# Autodesk Inventor assembly: Сборка
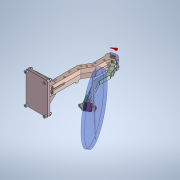
[picture p0: Inventor's stored thumbnail of the model, 180x180]
Saved by Autodesk Inventor 2021.2 (Build 252289000, 289)
## iProperties
Created: 2024-10-29
Part Number: Сборка
Document SubType Name: Assembly
Designer: barko
Mass: 1383.59 g
Surface Area: 2828.64 cm^2
Volume: 1218.78 cm^3
Density: 1.13522 g/cm^3
Author: barko
## Documents named in this file (30)
- C:\Users\barko\Desktop\Daniil\MIET\PID_controller\Mechanics\3D_model\Сборка.iam
- C:\Users\barko\Desktop\Daniil\MIET\PID_controller\Mechanics\3D_model\Детали твёрдого тела\Ножка 1.ipt
- C:\Users\barko\Desktop\Daniil\MIET\PID_controller\Mechanics\3D_model\Детали твёрдого тела\Ножка 2.ipt
- C:\Users\barko\Desktop\Daniil\MIET\PID_controller\Mechanics\3D_model\Детали твёрдого тела\Скобка 1.ipt
- C:\Users\barko\Desktop\Daniil\MIET\PID_controller\Mechanics\3D_model\Детали твёрдого тела\Скобка 2.ipt
- C:\Users\barko\Desktop\Daniil\MIET\PID_controller\Mechanics\3D_model\Детали твёрдого тела\Фланец.ipt
- C:\Users\barko\Desktop\Daniil\MIET\PID_controller\Mechanics\3D_model\Детали твёрдого тела\Луч.ipt
- C:\Users\barko\Desktop\Daniil\MIET\PID_controller\Mechanics\3D_model\Детали твёрдого тела\Ложечка.ipt
- C:\Users\barko\Desktop\Daniil\MIET\PID_controller\Mechanics\3D_model\Моторчик.ipt
- C:\Users\barko\Desktop\Daniil\MIET\PID_controller\Mechanics\3D_model\Пропеллер.ipt
- C:\Users\barko\Documents\Inventor\Content Center Files\R2021\ru-RU\Nut GOST 15524-70\Гайка M4-6H ГОСТ 15524-70.ipt
- C:\Users\barko\Documents\Inventor\Content Center Files\R2021\ru-RU\GOST 11738-84\Винт M4-6gx20 ГОСТ 11738-84.ipt
- C:\Users\barko\Desktop\Daniil\MIET\PID_controller\Mechanics\3D_model\Подшипник.ipt
- C:\Users\barko\Documents\Inventor\Content Center Files\R2021\ru-RU\GOST 5915-70\Гайка M6-6H ГОСТ 5915-70(1).ipt
- C:\Users\barko\Documents\Inventor\Content Center Files\R2021\ru-RU\GOST 11738-84\Винт M6-6gx50 ГОСТ 11738-84.ipt
- C:\Users\barko\Documents\Inventor\Content Center Files\R2021\ru-RU\GOST 11371-78  A\Шайба 6 ГОСТ 11371-78.ipt
- C:\Users\barko\Documents\Inventor\Content Center Files\R2021\ru-RU\Washer 1 GOST 6402-78\Шайба 6Л ГОСТ 6402-78.ipt
- C:\Users\barko\Documents\Inventor\Content Center Files\R2021\ru-RU\GOST 17475-80 (2)\Винт 2.M6-6gx30 ГОСТ 17475-80.ipt
- C:\Users\barko\Documents\Inventor\Content Center Files\R2021\ru-RU\ISO 10642(1)\ISO 10642 - M3x8.ipt
- C:\Users\barko\Documents\Inventor\Content Center Files\R2021\ru-RU\ISO 10642(1)\ISO 10642 - M3x12.ipt
- C:\Users\barko\Desktop\Daniil\MIET\PID_controller\Mechanics\3D_model\Детали твёрдого тела\Вал насадка 1.ipt
- C:\Users\barko\Desktop\Daniil\MIET\PID_controller\Mechanics\3D_model\Метизы\Гайка M4-6H ГОСТ 11860-85.ipt
- C:\Users\barko\Desktop\Daniil\MIET\PID_controller\Mechanics\3D_model\Метизы\Шайба A 4 ГОСТ 6958-78.ipt
- C:\Users\barko\Desktop\Daniil\MIET\PID_controller\Mechanics\3D_model\Стрелочка.ipt
- C:\Users\barko\Documents\Inventor\Content Center Files\R2021\ru-RU\GOST 11738-84\Винт M4-6gx25 ГОСТ 11738-84.ipt
- C:\Users\barko\Documents\Inventor\Content Center Files\R2021\ru-RU\GOST 11738-84\Винт M6-6gx30 ГОСТ 11738-84.ipt
- C:\Users\barko\Desktop\Daniil\MIET\PID_controller\Mechanics\3D_model\Детали твёрдого тела\Вал стержень.ipt
- C:\Users\barko\Desktop\Daniil\MIET\PID_controller\Mechanics\3D_model\Детали твёрдого тела\Блок.ipt
- C:\Users\barko\Documents\Inventor\Content Center Files\R2021\ru-RU\GOST 11738-84\Винт M3-6gx30 ГОСТ 11738-84.ipt
- C:\Users\barko\Documents\Inventor\Content Center Files\R2021\ru-RU\GOST 5916-70\Гайка M3-6H ГОСТ 5916-70.ipt
## Components (78 placed, 29 different names)
1. Ножка 1:1 — Совмещение:1, Угол:1, Совмещение:62, Совмещение:64, Вставка:26, Совмещение:100, Совмещение:101, Совмещение:102, Совмещение:105, Совмещение:106, Совмещение:107, Совмещение:127, Совмещение:128, Совмещение:129, Совмещение:130, Совмещение:131, Совмещение:132, Совмещение:133, Совмещение:134, Совмещение:135, Совмещение:136, Совмещение:137, Совмещение:138, Совмещение:139, Совмещение:140, Совмещение:141, Совмещение:142, Совмещение:143, Совмещение:144, Совмещение:145, Совмещение:147, Совмещение:149, Совмещение:151, Совмещение:153, Совмещение:155, Совмещение:157, Совмещение:159, Совмещение:161
2. Ножка 2:1 — Совмещение:63, Совмещение:65, Совмещение:115, Совмещение:116, Совмещение:117, Совмещение:121, Совмещение:122, Совмещение:123, Совмещение:146, Совмещение:148, Совмещение:150, Совмещение:152, Совмещение:154, Совмещение:156, Совмещение:158, Совмещение:160, Совмещение:162
3. Скобка 1:1 — Совмещение:104, Совмещение:109
4. Скобка 2:1 — Совмещение:119, Совмещение:120
5. Фланец:1 — Совмещение:66, Совмещение:67, Совмещение:68, Совмещение:69, Совмещение:70, Совмещение:71, Совмещение:72, Совмещение:73, Совмещение:74, Совмещение:75, Совмещение:76, Совмещение:77, Вставка:6, Вставка:7, Вставка:8, Вставка:9, Заподлицо:2, Заподлицо:3, Заподлицо:4, Заподлицо:5
6. Луч:1 — Заподлицо:1, Совмещение:1, Угол:1, Совмещение:96, Угол:2, Совмещение:97, Заподлицо:6, Угол:3, Совмещение:110, Совмещение:111, Совмещение:112, Совмещение:114
7. Ложечка:1 — Совмещение:87, Совмещение:88, Совмещение:91, Совмещение:92, Совмещение:93, Совмещение:94, Совмещение:96, Угол:2, Совмещение:97, Заподлицо:6, Совмещение:98, Совмещение:99
8. Моторчик:1 — Вставка:2, Совмещение:98, Совмещение:99
9. Пропеллер:1 — Вставка:2
10. Подшипник:1 — Вставка:25, Вставка:26, Вставка:29
11. Подшипник:2 — Вставка:32, Вставка:34
12. Вал насадка 1:1 — Вставка:25, Вставка:32, Совмещение:125
13. Гайка M4-6H ГОСТ 11860-85:2
14. Стрелочка:1 — Угол:3
15. Шайба A 4 ГОСТ 6958-78:3 — Вставка:29, Вставка:33
16. Вал стержень:1 — Совмещение:125, Заподлицо:7
17. Гайка ГОСТ 15524-70 M4:6 — Вставка:33, Заподлицо:7
18. Блок:1 — Вставка:35, Вставка:36, Совмещение:126
19. Шайба A 4 ГОСТ 6958-78:4 — Вставка:34, Вставка:35
20. Гайка ГОСТ 15524-70 M4:7 — Вставка:36, Совмещение:126
21. Гайка ГОСТ 5916-70 M3:9 — Совмещение:161, Совмещение:162
22. Гайка ГОСТ 5916-70 M3:8 — Совмещение:159, Совмещение:160
23. Гайка ГОСТ 5916-70 M3:7 — Совмещение:157, Совмещение:158
24. Гайка ГОСТ 5916-70 M3:6 — Совмещение:155, Совмещение:156
25. Гайка ГОСТ 5916-70 M3:5 — Совмещение:153, Совмещение:154
26. Гайка ГОСТ 5916-70 M3:4 — Совмещение:151, Совмещение:152
27. Гайка ГОСТ 5916-70 M3:3 — Совмещение:149, Совмещение:150
28. Гайка ГОСТ 5916-70 M3:2 — Совмещение:147, Совмещение:148
29. Винт ГОСТ 11738-84 M 3x30:9 — Совмещение:143, Совмещение:144
30. Винт ГОСТ 11738-84 M 3x30:8 — Совмещение:141, Совмещение:142
31. Винт ГОСТ 11738-84 M 3x30:7 — Совмещение:139, Совмещение:140
32. Винт ГОСТ 11738-84 M 3x30:6 — Совмещение:137, Совмещение:138
33. Винт ГОСТ 11738-84 M 3x30:5 — Совмещение:135, Совмещение:136
34. Винт ГОСТ 11738-84 M 3x30:4 — Совмещение:133, Совмещение:134
35. Винт ГОСТ 11738-84 M 3x30:3 — Совмещение:131, Совмещение:132
36. Винт ГОСТ 11738-84 M 3x30:2 — Совмещение:129, Совмещение:130
37. Гайка ГОСТ 5916-70 M3:1 — Совмещение:145, Совмещение:146
38. Винт ГОСТ 11738-84 M 3x30:1 — Совмещение:127, Совмещение:128
39. Винт ГОСТ 11738-84 M 4x25:1 — Совмещение:103, Совмещение:104
40. Гайка ГОСТ 15524-70 M4:1 — Совмещение:100, Совмещение:101, Совмещение:102, Совмещение:103
41. Винт ГОСТ 11738-84 M 4x25:2 — Совмещение:113, Совмещение:114
42. Гайка ГОСТ 15524-70 M4:2 — Совмещение:110, Совмещение:111, Совмещение:112, Совмещение:113
43. Винт ГОСТ 11738-84 M 4x20:2 — Совмещение:108, Совмещение:109
44. Винт ГОСТ 11738-84 M 4x25:3 — Совмещение:118, Совмещение:119
45. Винт ГОСТ 11738-84 M 4x20:4 — Совмещение:120, Совмещение:124
46. Гайка ГОСТ 15524-70 M4:3 — Совмещение:115, Совмещение:116, Совмещение:117, Совмещение:118
47. Гайка ГОСТ 15524-70 M4:4 — Совмещение:105, Совмещение:106, Совмещение:107, Совмещение:108
48. Гайка ГОСТ 15524-70 M4:5 — Совмещение:121, Совмещение:122, Совмещение:123, Совмещение:124
49. Гайка ГОСТ 5915-70 M6:1 — Совмещение:69, Совмещение:72, Совмещение:73, Совмещение:80
50. Гайка ГОСТ 5915-70 M6:2 — Совмещение:71, Совмещение:74, Совмещение:75, Совмещение:81
51. Гайка ГОСТ 5915-70 M6:3 — Совмещение:70, Совмещение:76, Совмещение:77, Совмещение:79
52. Гайка ГОСТ 5915-70 M6:4 — Совмещение:66, Совмещение:67, Совмещение:68, Совмещение:78
53. Винт ГОСТ 11738-84 M 6x50:1 — Совмещение:64, Совмещение:79
54. Винт ГОСТ 11738-84 M 6x30:1 — Совмещение:63, Совмещение:80
55. Винт ГОСТ 11738-84 M 6x30:2 — Совмещение:62, Совмещение:78
56. Винт ГОСТ 11738-84 M 6x50:2 — Совмещение:65, Совмещение:81
57. Шайба  ГОСТ 11371-78 6,4:1 — Вставка:6, Вставка:10
58. Шайба  ГОСТ 11371-78 6,4:2 — Вставка:7, Вставка:11
59. Шайба  ГОСТ 11371-78 6,4:3 — Вставка:8, Вставка:13
60. Шайба  ГОСТ 11371-78 6,4:4 — Вставка:9, Вставка:12
61. Шайба 1 ГОСТ 6402-78 6Л:1 — Вставка:10, Вставка:16
62. Шайба 1 ГОСТ 6402-78 6Л:2 — Вставка:11, Вставка:15
63. Шайба 1 ГОСТ 6402-78 6Л:3 — Вставка:12, Вставка:17
64. Шайба 1 ГОСТ 6402-78 6Л:4 — Вставка:13, Вставка:14
65. Гайка ГОСТ 5915-70 M6:5 — Вставка:14, Совмещение:85
66. Гайка ГОСТ 5915-70 M6:6 — Вставка:15, Совмещение:84
67. Гайка ГОСТ 5915-70 M6:7 — Вставка:16, Совмещение:82
68. Гайка ГОСТ 5915-70 M6:8 — Вставка:17, Совмещение:83
69. Винт 2 ГОСТ 17475-80 M6 x 30:1 — Совмещение:82, Заподлицо:3
70. Винт 2 ГОСТ 17475-80 M6 x 30:2 — Совмещение:83, Заподлицо:2
71. Винт 2 ГОСТ 17475-80 M6 x 30:3 — Совмещение:85, Заподлицо:5
72. Винт 2 ГОСТ 17475-80 M6 x 30:4 — Совмещение:84, Заподлицо:4
73. ISO 10642 M3x12:2 — Совмещение:87
74. ISO 10642 M3x12:3 — Совмещение:88
75. ISO 10642 M3x8:1 — Совмещение:91
76. ISO 10642 M3x8:2 — Совмещение:92
77. ISO 10642 M3x8:3 — Совмещение:93
78. ISO 10642 M3x8:4 — Совмещение:94
## Relationships (129: Mate 98, Insert 21, Flush 7, Angle 3)
- Вставка:2 [Insert] (2 mm): Моторчик:1 ↔ Пропеллер:1
- Заподлицо:1 [Flush]: Луч:1
- Совмещение:1 [Mate]: Ножка 1:1 ↔ Луч:1
- Угол:1 [Angle] (0 deg): Ножка 1:1 ↔ Луч:1
- Совмещение:62 [Mate]: Ножка 1:1 ↔ Винт ГОСТ 11738-84 M 6x30:2
- Совмещение:63 [Mate]: Ножка 2:1 ↔ Винт ГОСТ 11738-84 M 6x30:1
- Совмещение:64 [Mate]: Ножка 1:1 ↔ Винт ГОСТ 11738-84 M 6x50:1
- Совмещение:65 [Mate]: Ножка 2:1 ↔ Винт ГОСТ 11738-84 M 6x50:2
- Совмещение:66 [Mate]: Фланец:1 ↔ Гайка ГОСТ 5915-70 M6:4
- Совмещение:67 [Mate]: Фланец:1 ↔ Гайка ГОСТ 5915-70 M6:4
- Совмещение:68 [Mate]: Фланец:1 ↔ Гайка ГОСТ 5915-70 M6:4
- Совмещение:69 [Mate]: Фланец:1 ↔ Гайка ГОСТ 5915-70 M6:1
- Совмещение:70 [Mate]: Фланец:1 ↔ Гайка ГОСТ 5915-70 M6:3
- Совмещение:71 [Mate]: Фланец:1 ↔ Гайка ГОСТ 5915-70 M6:2
- Совмещение:72 [Mate]: Фланец:1 ↔ Гайка ГОСТ 5915-70 M6:1
- Совмещение:73 [Mate]: Фланец:1 ↔ Гайка ГОСТ 5915-70 M6:1
- Совмещение:74 [Mate]: Фланец:1 ↔ Гайка ГОСТ 5915-70 M6:2
- Совмещение:75 [Mate]: Фланец:1 ↔ Гайка ГОСТ 5915-70 M6:2
- Совмещение:76 [Mate]: Фланец:1 ↔ Гайка ГОСТ 5915-70 M6:3
- Совмещение:77 [Mate]: Фланец:1 ↔ Гайка ГОСТ 5915-70 M6:3
- Совмещение:78 [Mate]: Гайка ГОСТ 5915-70 M6:4 ↔ Винт ГОСТ 11738-84 M 6x30:2
- Совмещение:79 [Mate]: Гайка ГОСТ 5915-70 M6:3 ↔ Винт ГОСТ 11738-84 M 6x50:1
- Совмещение:80 [Mate]: Гайка ГОСТ 5915-70 M6:1 ↔ Винт ГОСТ 11738-84 M 6x30:1
- Совмещение:81 [Mate]: Гайка ГОСТ 5915-70 M6:2 ↔ Винт ГОСТ 11738-84 M 6x50:2
- Вставка:6 [Insert]: Фланец:1 ↔ Шайба  ГОСТ 11371-78 6,4:1
- Вставка:7 [Insert]: Фланец:1 ↔ Шайба  ГОСТ 11371-78 6,4:2
- Вставка:8 [Insert]: Фланец:1 ↔ Шайба  ГОСТ 11371-78 6,4:3
- Вставка:9 [Insert]: Фланец:1 ↔ Шайба  ГОСТ 11371-78 6,4:4
- Вставка:10 [Insert]: Шайба  ГОСТ 11371-78 6,4:1 ↔ Шайба 1 ГОСТ 6402-78 6Л:1
- Вставка:11 [Insert]: Шайба  ГОСТ 11371-78 6,4:2 ↔ Шайба 1 ГОСТ 6402-78 6Л:2
- Вставка:12 [Insert]: Шайба  ГОСТ 11371-78 6,4:4 ↔ Шайба 1 ГОСТ 6402-78 6Л:3
- Вставка:13 [Insert]: Шайба  ГОСТ 11371-78 6,4:3 ↔ Шайба 1 ГОСТ 6402-78 6Л:4
- Вставка:14 [Insert]: Шайба 1 ГОСТ 6402-78 6Л:4 ↔ Гайка ГОСТ 5915-70 M6:5
- Вставка:15 [Insert]: Шайба 1 ГОСТ 6402-78 6Л:2 ↔ Гайка ГОСТ 5915-70 M6:6
- Вставка:16 [Insert]: Шайба 1 ГОСТ 6402-78 6Л:1 ↔ Гайка ГОСТ 5915-70 M6:7
- Вставка:17 [Insert]: Шайба 1 ГОСТ 6402-78 6Л:3 ↔ Гайка ГОСТ 5915-70 M6:8
- Совмещение:82 [Mate]: Гайка ГОСТ 5915-70 M6:7 ↔ Винт 2 ГОСТ 17475-80 M6 x 30:1
- Совмещение:83 [Mate]: Гайка ГОСТ 5915-70 M6:8 ↔ Винт 2 ГОСТ 17475-80 M6 x 30:2
- Совмещение:84 [Mate]: Гайка ГОСТ 5915-70 M6:6 ↔ Винт 2 ГОСТ 17475-80 M6 x 30:4
- Совмещение:85 [Mate]: Гайка ГОСТ 5915-70 M6:5 ↔ Винт 2 ГОСТ 17475-80 M6 x 30:3
- Заподлицо:2 [Flush] (9 mm): Фланец:1 ↔ Винт 2 ГОСТ 17475-80 M6 x 30:2
- Заподлицо:3 [Flush] (9 mm): Фланец:1 ↔ Винт 2 ГОСТ 17475-80 M6 x 30:1
- Заподлицо:4 [Flush] (9 mm): Фланец:1 ↔ Винт 2 ГОСТ 17475-80 M6 x 30:4
- Заподлицо:5 [Flush] (9 mm): Фланец:1 ↔ Винт 2 ГОСТ 17475-80 M6 x 30:3
- Совмещение:87 [Mate]: Ложечка:1 ↔ ISO 10642 M3x12:2
- Совмещение:88 [Mate]: Ложечка:1 ↔ ISO 10642 M3x12:3
- Совмещение:91 [Mate]: Ложечка:1 ↔ ISO 10642 M3x8:1
- Совмещение:92 [Mate]: Ложечка:1 ↔ ISO 10642 M3x8:2
- Совмещение:93 [Mate]: Ложечка:1 ↔ ISO 10642 M3x8:3
- Совмещение:94 [Mate]: Ложечка:1 ↔ ISO 10642 M3x8:4
- Совмещение:96 [Mate]: Луч:1 ↔ Ложечка:1
- Угол:2 [Angle] (180 deg): Луч:1 ↔ Ложечка:1
- Совмещение:97 [Mate]: Луч:1 ↔ Ложечка:1
- Заподлицо:6 [Flush]: Луч:1 ↔ Ложечка:1
- Совмещение:98 [Mate]: Ложечка:1 ↔ Моторчик:1
- Совмещение:99 [Mate]: Ложечка:1 ↔ Моторчик:1
- Вставка:25 [Insert]: Подшипник:1 ↔ Вал насадка 1:1
- Вставка:26 [Insert]: Ножка 1:1 ↔ Подшипник:1
- Угол:3 [Angle] (90 deg): Луч:1 ↔ Стрелочка:1
- Совмещение:100 [Mate]: Ножка 1:1 ↔ Гайка ГОСТ 15524-70 M4:1
- Совмещение:101 [Mate]: Ножка 1:1 ↔ Гайка ГОСТ 15524-70 M4:1
- Совмещение:102 [Mate]: Ножка 1:1 ↔ Гайка ГОСТ 15524-70 M4:1
- Совмещение:103 [Mate]: Винт ГОСТ 11738-84 M 4x25:1 ↔ Гайка ГОСТ 15524-70 M4:1
- Совмещение:104 [Mate]: Скобка 1:1 ↔ Винт ГОСТ 11738-84 M 4x25:1
- Совмещение:105 [Mate]: Ножка 1:1 ↔ Гайка ГОСТ 15524-70 M4:4
- Совмещение:106 [Mate]: Ножка 1:1 ↔ Гайка ГОСТ 15524-70 M4:4
- Совмещение:107 [Mate]: Ножка 1:1 ↔ Гайка ГОСТ 15524-70 M4:4
- Совмещение:108 [Mate]: Винт ГОСТ 11738-84 M 4x20:2 ↔ Гайка ГОСТ 15524-70 M4:4
- Совмещение:109 [Mate]: Скобка 1:1 ↔ Винт ГОСТ 11738-84 M 4x20:2
- Совмещение:110 [Mate]: Луч:1 ↔ Гайка ГОСТ 15524-70 M4:2
- Совмещение:111 [Mate]: Луч:1 ↔ Гайка ГОСТ 15524-70 M4:2
- Совмещение:112 [Mate]: Луч:1 ↔ Гайка ГОСТ 15524-70 M4:2
- Совмещение:113 [Mate]: Винт ГОСТ 11738-84 M 4x25:2 ↔ Гайка ГОСТ 15524-70 M4:2
- Совмещение:114 [Mate]: Луч:1 ↔ Винт ГОСТ 11738-84 M 4x25:2
- Совмещение:115 [Mate]: Ножка 2:1 ↔ Гайка ГОСТ 15524-70 M4:3
- Совмещение:116 [Mate]: Ножка 2:1 ↔ Гайка ГОСТ 15524-70 M4:3
- Совмещение:117 [Mate]: Ножка 2:1 ↔ Гайка ГОСТ 15524-70 M4:3
- Совмещение:118 [Mate]: Винт ГОСТ 11738-84 M 4x25:3 ↔ Гайка ГОСТ 15524-70 M4:3
- Совмещение:119 [Mate]: Скобка 2:1 ↔ Винт ГОСТ 11738-84 M 4x25:3
- Совмещение:120 [Mate]: Скобка 2:1 ↔ Винт ГОСТ 11738-84 M 4x20:4
- Совмещение:121 [Mate]: Ножка 2:1 ↔ Гайка ГОСТ 15524-70 M4:5
- Совмещение:122 [Mate]: Ножка 2:1 ↔ Гайка ГОСТ 15524-70 M4:5
- Совмещение:123 [Mate]: Ножка 2:1 ↔ Гайка ГОСТ 15524-70 M4:5
- Совмещение:124 [Mate]: Винт ГОСТ 11738-84 M 4x20:4 ↔ Гайка ГОСТ 15524-70 M4:5
- Вставка:29 [Insert]: Подшипник:1 ↔ Шайба A 4 ГОСТ 6958-78:3
- Вставка:32 [Insert]: Подшипник:2 ↔ Вал насадка 1:1
- Совмещение:125 [Mate]: Вал насадка 1:1 ↔ Вал стержень:1
- Вставка:33 [Insert]: Шайба A 4 ГОСТ 6958-78:3 ↔ Гайка ГОСТ 15524-70 M4:6
- Заподлицо:7 [Flush] (-2 mm): Вал стержень:1 ↔ Гайка ГОСТ 15524-70 M4:6
- Вставка:34 [Insert]: Подшипник:2 ↔ Шайба A 4 ГОСТ 6958-78:4
- Вставка:35 [Insert]: Блок:1 ↔ Шайба A 4 ГОСТ 6958-78:4
- Вставка:36 [Insert]: Блок:1 ↔ Гайка ГОСТ 15524-70 M4:7
- Совмещение:126 [Mate]: Блок:1 ↔ Гайка ГОСТ 15524-70 M4:7
- Совмещение:127 [Mate]: Ножка 1:1 ↔ Винт ГОСТ 11738-84 M 3x30:1
- Совмещение:128 [Mate]: Ножка 1:1 ↔ Винт ГОСТ 11738-84 M 3x30:1
- Совмещение:129 [Mate]: Ножка 1:1 ↔ Винт ГОСТ 11738-84 M 3x30:2
- Совмещение:130 [Mate]: Ножка 1:1 ↔ Винт ГОСТ 11738-84 M 3x30:2
- Совмещение:131 [Mate]: Ножка 1:1 ↔ Винт ГОСТ 11738-84 M 3x30:3
- Совмещение:132 [Mate]: Ножка 1:1 ↔ Винт ГОСТ 11738-84 M 3x30:3
- Совмещение:133 [Mate]: Ножка 1:1 ↔ Винт ГОСТ 11738-84 M 3x30:4
- Совмещение:134 [Mate]: Ножка 1:1 ↔ Винт ГОСТ 11738-84 M 3x30:4
- Совмещение:135 [Mate]: Ножка 1:1 ↔ Винт ГОСТ 11738-84 M 3x30:5
- Совмещение:136 [Mate]: Ножка 1:1 ↔ Винт ГОСТ 11738-84 M 3x30:5
- Совмещение:137 [Mate]: Ножка 1:1 ↔ Винт ГОСТ 11738-84 M 3x30:6
- Совмещение:138 [Mate]: Ножка 1:1 ↔ Винт ГОСТ 11738-84 M 3x30:6
- Совмещение:139 [Mate]: Ножка 1:1 ↔ Винт ГОСТ 11738-84 M 3x30:7
- Совмещение:140 [Mate]: Ножка 1:1 ↔ Винт ГОСТ 11738-84 M 3x30:7
- Совмещение:141 [Mate]: Ножка 1:1 ↔ Винт ГОСТ 11738-84 M 3x30:8
- Совмещение:142 [Mate]: Ножка 1:1 ↔ Винт ГОСТ 11738-84 M 3x30:8
- Совмещение:143 [Mate]: Ножка 1:1 ↔ Винт ГОСТ 11738-84 M 3x30:9
- Совмещение:144 [Mate]: Ножка 1:1 ↔ Винт ГОСТ 11738-84 M 3x30:9
- Совмещение:145 [Mate]: Ножка 1:1 ↔ Гайка ГОСТ 5916-70 M3:1
- Совмещение:146 [Mate]: Ножка 2:1 ↔ Гайка ГОСТ 5916-70 M3:1
- Совмещение:147 [Mate]: Ножка 1:1 ↔ Гайка ГОСТ 5916-70 M3:2
- Совмещение:148 [Mate]: Ножка 2:1 ↔ Гайка ГОСТ 5916-70 M3:2
- Совмещение:149 [Mate]: Ножка 1:1 ↔ Гайка ГОСТ 5916-70 M3:3
- Совмещение:150 [Mate]: Ножка 2:1 ↔ Гайка ГОСТ 5916-70 M3:3
- Совмещение:151 [Mate]: Ножка 1:1 ↔ Гайка ГОСТ 5916-70 M3:4
- Совмещение:152 [Mate]: Ножка 2:1 ↔ Гайка ГОСТ 5916-70 M3:4
- Совмещение:153 [Mate]: Ножка 1:1 ↔ Гайка ГОСТ 5916-70 M3:5
- Совмещение:154 [Mate]: Ножка 2:1 ↔ Гайка ГОСТ 5916-70 M3:5
- Совмещение:155 [Mate]: Ножка 1:1 ↔ Гайка ГОСТ 5916-70 M3:6
- Совмещение:156 [Mate]: Ножка 2:1 ↔ Гайка ГОСТ 5916-70 M3:6
- Совмещение:157 [Mate]: Ножка 1:1 ↔ Гайка ГОСТ 5916-70 M3:7
- Совмещение:158 [Mate]: Ножка 2:1 ↔ Гайка ГОСТ 5916-70 M3:7
- Совмещение:159 [Mate]: Ножка 1:1 ↔ Гайка ГОСТ 5916-70 M3:8
- Совмещение:160 [Mate]: Ножка 2:1 ↔ Гайка ГОСТ 5916-70 M3:8
- Совмещение:161 [Mate]: Ножка 1:1 ↔ Гайка ГОСТ 5916-70 M3:9
- Совмещение:162 [Mate]: Ножка 2:1 ↔ Гайка ГОСТ 5916-70 M3:9
